# Autodesk Inventor assembly: micro-switch-assembly
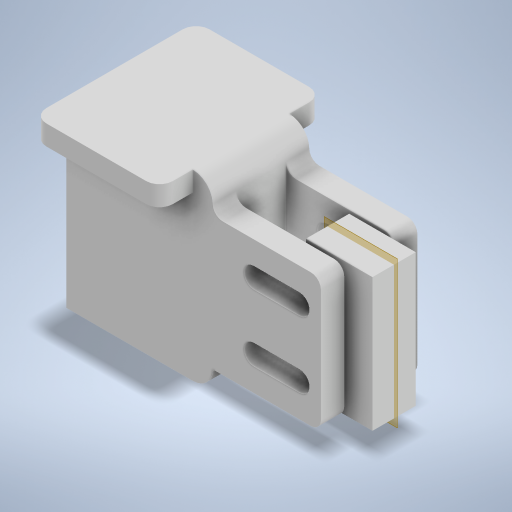
[picture p0: Inventor's stored thumbnail of the model, 512x512]
Saved by Autodesk Inventor 2024 (Build 280153000, 153)
## iProperties
Created: 2024-05-14
Part Number: micro-switch-assembly
Document SubType Name: Assembly
Designer: MaartenGeorgesBuelen
Author: MaartenGeorgesBuelen
## Documents named in this file (3)
- C:\Users\MaartenGeorgesBuelen\Documents\Inventor\robot arm\hardware\micro-switch-assembly.iam
- C:\Users\MaartenGeorgesBuelen\Documents\Inventor\robot arm\hardware\micro-switch.ipt
- C:\Users\MaartenGeorgesBuelen\Documents\Inventor\robot arm\hardware\micro-switch-holder.ipt
## Components (2 placed, 2 different names)
1. micro-switch:1 — Flush:1
2. micro-switch-holder:1 — Flush:1
## Relationships (1: Flush 1)
- Flush:1: micro-switch:1 ↔ micro-switch-holder:1
